# Autodesk Inventor assembly: 202.001.01_Schieberbetaetigung
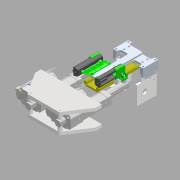
[picture p0: Inventor's stored thumbnail of the model, 180x180]
Saved by Autodesk Inventor 2021 (Build 250183000, 183)
## iProperties
Created: 2021-11-14
Part Number: 202.001.01_Schieberbetaetigung
Document SubType Name: Assembly
Designer: Oliver Ungerer
KODE_ZEICHNUNGSNUMMER: TFVEM_110M
BENENNUNG: Fuehrung Schieber
BEARBEITER_NAME: Ungerer O.
MASSE: 2.190774
PDMREV: 0.0+
PDMRL: Entwicklung
PROI_REVISION: 0
PROI_VERSION: 0+
PROI_RELEASE: Entwicklung
PTC_MODIFIED: True
PROI_CREATED_BY: Kantioler_adm
PROI_CREATED_ON: 07.03.2008 12:11:19
PROI_LOCATION: Root-Ordner/Pro_stds/Start_Files
MATERIALART: -
EINHEIT: ST
HERSTELLER_PREIS: 0.0
PRUEFER_NAME: Uo
PTC_ORGANIZATION_ID: Durst
PTC_WM_REVISION: 0
PTC_WM_ITERATION: 0
PTC_WM_VERSION: 0.0
PTC_WM_LIFECYCLE_STATE: Entwicklung
PTC_WM_LIFECYCLE: 02 Durst
PTC_WM_CREATED_BY: Oliver Ungerer (oungerer: Durst)
PTC_WM_CREATED_ON: 01.08.21
PTC_WM_MODIFIED_BY: Oliver Ungerer (oungerer: Durst)
PTC_WM_MODIFIED_ON: 01.08.21
AEND_INDEX: 0
VERSION: 0
STATUS: 0.0
Author: Oliver Ungerer
## Documents named in this file (20)
- E:\Dokumente\MCI-Mechatronik\Master\Semester_3\Projekt2_CAD\102_Vereinzelung\202.001.01_Schieberbetaetigung.iam
- E:\Dokumente\MCI-Mechatronik\Master\Semester_3\Projekt2_CAD\102_Vereinzelung\0001_IGUS_SCHIENE.ipt
- E:\Dokumente\MCI-Mechatronik\Master\Semester_3\Projekt2_CAD\102_Vereinzelung\1346134.ipt
- E:\Dokumente\MCI-Mechatronik\Master\Semester_3\Projekt2_CAD\102_Vereinzelung\TFVEM_10100.ipt
- E:\Dokumente\MCI-Mechatronik\Master\Semester_3\Projekt2_CAD\102_Vereinzelung\TFVEM_1106.ipt
- E:\Dokumente\MCI-Mechatronik\Master\Semester_3\Projekt2_CAD\102_Vereinzelung\TFVEM_1101.ipt
- E:\Dokumente\MCI-Mechatronik\Master\Semester_3\Projekt2_CAD\102_Vereinzelung\TFVEM_10102.ipt
- E:\Dokumente\MCI-Mechatronik\Master\Semester_3\Projekt2_CAD\102_Vereinzelung\TFVEM_10103.ipt
- E:\Dokumente\MCI-Mechatronik\Master\Semester_3\Projekt2_CAD\102_Vereinzelung\TFVEM_10104.ipt
- E:\Dokumente\MCI-Mechatronik\Master\Semester_3\Projekt2_CAD\102_Vereinzelung\202.001.02_Kraftlimitierung.iam
- E:\Dokumente\MCI-Mechatronik\Master\Semester_3\Projekt2_CAD\102_Vereinzelung\202.001.03_Kraftlimitierung.iam
- E:\Dokumente\MCI-Mechatronik\Master\Semester_3\Projekt2_CAD\102_Vereinzelung\CAHB-10-B1A-050158-AAAA0A-000.iam
- E:\Dokumente\MCI-Mechatronik\Master\Semester_3\Projekt2_CAD\102_Vereinzelung\TFVEM_10105.ipt
- E:\Dokumente\MCI-Mechatronik\Master\Semester_3\Projekt2_CAD\102_Vereinzelung\TFVEM_1009.ipt
- E:\Dokumente\MCI-Mechatronik\Master\Semester_3\Projekt2_CAD\102_Vereinzelung\1237347.ipt
- E:\Dokumente\MCI-Mechatronik\Master\Semester_3\Projekt2_CAD\102_Vereinzelung\1126405.ipt
- E:\Dokumente\MCI-Mechatronik\Master\Semester_3\Projekt2_CAD\102_Vereinzelung\1126767.ipt
- E:\Dokumente\MCI-Mechatronik\Master\Semester_3\Projekt2_CAD\102_Vereinzelung\202.001.04_Zapfen_Aktor.ipt
- E:\Dokumente\MCI-Mechatronik\Master\Semester_3\Projekt2_CAD\102_Vereinzelung\202.001.05_Zapfen_Aktor_Auflage.ipt
- E:\Dokumente\MCI-Mechatronik\Master\Semester_3\Projekt2_CAD\102_Vereinzelung\202.001.05_Anbindung_Aktor.ipt
## Components (31 placed, 20 different names)
1. 0001_IGUS_SCHIENE — Fluchtend:1, Passend:15, Winkel:1, Passend:20, Winkel:2, Fluchtend:2, Passend:21, Winkel:3, Passend:23, Winkel:4, Fluchtend:69, Winkel:5
2. 1346134 — Fluchtend:1, Passend:15, Winkel:1, Passend:16, Passend:17, Passend:18, Passend:19
3. 1346134:1 — Passend:22, Passend:23, Winkel:4, Passend:24, Passend:25, Passend:26
4. 1346134:2 — Fluchtend:2, Passend:21, Winkel:3, Passend:22, Passend:30, Passend:32
5. 1346134:3 — Passend:19, Passend:20, Winkel:2, Passend:31
6. TFVEM_10100 — Passend:16, Passend:17, Passend:18, Passend:27, Passend:29
7. TFVEM_1106 — Passend:27, Passend:28, Passend:29, Passend:36, Passend:37, Passend:38, Passend:48, Passend:49, Passend:50
8. TFVEM_1101 — Passend:30, Passend:31, Passend:32, Passend:33, Passend:34, Passend:35, Passend:45, Passend:46, Passend:47
9. TFVEM_10100:1 — Passend:24, Passend:25, Passend:26, Passend:28
10. TFVEM_10102 — Passend:36, Passend:37, Passend:38, Passend:42, Passend:43, Passend:44
11. TFVEM_10103 — Passend:42, Passend:43, Passend:44
12. TFVEM_10102:1 — Passend:33, Passend:34, Passend:35, Passend:39, Passend:40, Passend:41
13. TFVEM_10104 — Passend:39, Passend:40, Passend:41
14. 202.001.02_Kraftlimitierung [sub-assembly] — Passend:45, Passend:46, Passend:47, Passend:51, Passend:52, Passend:53, Passend:54
15. 202.001.03_Kraftlimitierung [sub-assembly] — Passend:48, Passend:49, Passend:50, Passend:59, Passend:60, Passend:62
16. 502.001.01_Linearaktor [sub-assembly] — Passend:1, Passend:2, Fluchtend:70, Passend:70
17. CAHB-10-B1A-050158-AAAA0A-000:2 [sub-assembly] — Fluchtend:69, Passend:67, Winkel:5, Passend:68, Passend:69, Fluchtend:70
18. TFVEM_10105 — Passend:59, Passend:60, Passend:61, Passend:63, Passend:64, Passend:65, Passend:67
19. TFVEM_1009 — Passend:51, Passend:52, Passend:55, Passend:56, Passend:57, Passend:70
20. 1237347 — Passend:55, Passend:56, Passend:58
21. 1237347:1 — Passend:63, Passend:64, Passend:66
22. 1126405 — Passend:65, Passend:66
23. 1126405:1 — Passend:57, Passend:58
24. 1126767 — Passend:53, Passend:54
25. 1126767:1 — Passend:61, Passend:62
26. 202.001.04_Zapfen_Aktor:1 — Passend:7, Passend:8, Passend:68, Passend:69
27. 202.001.04_Zapfen_Aktor:2 — Passend:1, Passend:2, Passend:5, Passend:6
28. 202.001.05_Zapfen_Aktor_Auflage:3 — Passend:7, Passend:8
29. 202.001.05_Zapfen_Aktor_Auflage:4 — Passend:5, Passend:6
30. 202.001.05_Anbindung_Aktor:1
31. 202.001.05_Anbindung_Aktor:2
## Relationships (77: Mate 68, Angle 5, Flush 4)
- Passend:1 [Mate] (1 mm): 502.001.01_Linearaktor ↔ 202.001.04_Zapfen_Aktor:2
- Passend:2 [Mate]: 502.001.01_Linearaktor ↔ 202.001.04_Zapfen_Aktor:2
- Passend:5 [Mate]: 202.001.04_Zapfen_Aktor:2 ↔ 202.001.05_Zapfen_Aktor_Auflage:4
- Passend:6 [Mate]: 202.001.04_Zapfen_Aktor:2 ↔ 202.001.05_Zapfen_Aktor_Auflage:4
- Passend:7 [Mate]: 202.001.04_Zapfen_Aktor:1 ↔ 202.001.05_Zapfen_Aktor_Auflage:3
- Passend:8 [Mate]: 202.001.04_Zapfen_Aktor:1 ↔ 202.001.05_Zapfen_Aktor_Auflage:3
- [Mate]: 202.001.04_Zapfen_Aktor:2 ↔ 202.001.05_Anbindung_Aktor:1
- [Mate]: 202.001.04_Zapfen_Aktor:2 ↔ 202.001.05_Anbindung_Aktor:1
- [Mate]: 202.001.04_Zapfen_Aktor:1 ↔ 202.001.05_Anbindung_Aktor:1
- [Mate]: 202.001.05_Zapfen_Aktor_Auflage:4 ↔ 202.001.05_Anbindung_Aktor:2
- [Mate]: 202.001.05_Zapfen_Aktor_Auflage:3 ↔ 202.001.05_Anbindung_Aktor:2
- [Mate]: 202.001.05_Zapfen_Aktor_Auflage:4 ↔ 202.001.05_Anbindung_Aktor:2
- Fluchtend:1 [Flush] (0.5 mm): 0001_IGUS_SCHIENE ↔ 1346134
- Passend:15 [Mate]: 0001_IGUS_SCHIENE ↔ 1346134
- Winkel:1 [Angle] (0 deg): 0001_IGUS_SCHIENE ↔ 1346134
- Passend:16 [Mate]: 1346134 ↔ TFVEM_10100
- Passend:17 [Mate]: 1346134 ↔ TFVEM_10100
- Passend:18 [Mate]: 1346134 ↔ TFVEM_10100
- Passend:19 [Mate] (51 mm): 1346134 ↔ 1346134:3
- Passend:20 [Mate]: 0001_IGUS_SCHIENE ↔ 1346134:3
- Winkel:2 [Angle] (0 deg): 0001_IGUS_SCHIENE ↔ 1346134:3
- Fluchtend:2 [Flush] (0.5 mm): 0001_IGUS_SCHIENE ↔ 1346134:2
- Passend:21 [Mate]: 0001_IGUS_SCHIENE ↔ 1346134:2
- Winkel:3 [Angle] (0 deg): 0001_IGUS_SCHIENE ↔ 1346134:2
- Passend:22 [Mate] (51 mm): 1346134:1 ↔ 1346134:2
- Passend:23 [Mate]: 0001_IGUS_SCHIENE ↔ 1346134:1
- Winkel:4 [Angle] (0 deg): 0001_IGUS_SCHIENE ↔ 1346134:1
- Passend:24 [Mate]: 1346134:1 ↔ TFVEM_10100:1
- Passend:25 [Mate]: 1346134:1 ↔ TFVEM_10100:1
- Passend:26 [Mate]: 1346134:1 ↔ TFVEM_10100:1
- Passend:27 [Mate]: TFVEM_10100 ↔ TFVEM_1106
- Passend:28 [Mate]: TFVEM_1106 ↔ TFVEM_10100:1
- Passend:29 [Mate]: TFVEM_10100 ↔ TFVEM_1106
- Passend:30 [Mate]: 1346134:2 ↔ TFVEM_1101
- Passend:31 [Mate]: 1346134:3 ↔ TFVEM_1101
- Passend:32 [Mate]: 1346134:2 ↔ TFVEM_1101
- Passend:33 [Mate]: TFVEM_1101 ↔ TFVEM_10102:1
- Passend:34 [Mate]: TFVEM_1101 ↔ TFVEM_10102:1
- Passend:35 [Mate]: TFVEM_1101 ↔ TFVEM_10102:1
- Passend:36 [Mate]: TFVEM_1106 ↔ TFVEM_10102
- Passend:37 [Mate]: TFVEM_1106 ↔ TFVEM_10102
- Passend:38 [Mate]: TFVEM_1106 ↔ TFVEM_10102
- Passend:39 [Mate]: TFVEM_10102:1 ↔ TFVEM_10104
- Passend:40 [Mate]: TFVEM_10102:1 ↔ TFVEM_10104
- Passend:41 [Mate]: TFVEM_10102:1 ↔ TFVEM_10104
- Passend:42 [Mate]: TFVEM_10102 ↔ TFVEM_10103
- Passend:43 [Mate]: TFVEM_10102 ↔ TFVEM_10103
- Passend:44 [Mate]: TFVEM_10102 ↔ TFVEM_10103
- Passend:45 [Mate]: TFVEM_1101 ↔ 202.001.02_Kraftlimitierung
- Passend:46 [Mate]: TFVEM_1101 ↔ 202.001.02_Kraftlimitierung
- Passend:47 [Mate]: TFVEM_1101 ↔ 202.001.02_Kraftlimitierung
- Passend:48 [Mate]: TFVEM_1106 ↔ 202.001.03_Kraftlimitierung
- Passend:49 [Mate]: TFVEM_1106 ↔ 202.001.03_Kraftlimitierung
- Passend:50 [Mate]: TFVEM_1106 ↔ 202.001.03_Kraftlimitierung
- Passend:51 [Mate]: 202.001.02_Kraftlimitierung ↔ TFVEM_1009
- Passend:52 [Mate]: 202.001.02_Kraftlimitierung ↔ TFVEM_1009
- Passend:53 [Mate]: 202.001.02_Kraftlimitierung ↔ 1126767
- Passend:54 [Mate]: 202.001.02_Kraftlimitierung ↔ 1126767
- Passend:55 [Mate]: TFVEM_1009 ↔ 1237347
- Passend:56 [Mate]: TFVEM_1009 ↔ 1237347
- Passend:57 [Mate]: TFVEM_1009 ↔ 1126405:1
- Passend:58 [Mate]: 1237347 ↔ 1126405:1
- Passend:59 [Mate]: 202.001.03_Kraftlimitierung ↔ TFVEM_10105
- Passend:60 [Mate]: 202.001.03_Kraftlimitierung ↔ TFVEM_10105
- Passend:61 [Mate]: TFVEM_10105 ↔ 1126767:1
- Passend:62 [Mate]: 202.001.03_Kraftlimitierung ↔ 1126767:1
- Passend:63 [Mate]: TFVEM_10105 ↔ 1237347:1
- Passend:64 [Mate]: TFVEM_10105 ↔ 1237347:1
- Passend:65 [Mate]: TFVEM_10105 ↔ 1126405
- Passend:66 [Mate]: 1237347:1 ↔ 1126405
- Fluchtend:69 [Flush] (6 mm): 0001_IGUS_SCHIENE ↔ CAHB-10-B1A-050158-AAAA0A-000:2
- Passend:67 [Mate]: CAHB-10-B1A-050158-AAAA0A-000:2 ↔ TFVEM_10105
- Winkel:5 [Angle] (0 deg): 0001_IGUS_SCHIENE ↔ CAHB-10-B1A-050158-AAAA0A-000:2
- Passend:68 [Mate]: CAHB-10-B1A-050158-AAAA0A-000:2 ↔ 202.001.04_Zapfen_Aktor:1
- Passend:69 [Mate] (1 mm): CAHB-10-B1A-050158-AAAA0A-000:2 ↔ 202.001.04_Zapfen_Aktor:1
- Fluchtend:70 [Flush]: 502.001.01_Linearaktor ↔ CAHB-10-B1A-050158-AAAA0A-000:2
- Passend:70 [Mate]: 502.001.01_Linearaktor ↔ TFVEM_1009
## Named parameters: d8_d2 = 0 mm, d9_d3 = 0 mm, d10_d4 = 0 mm, d11_d6 = 0 mm, d12_d7 = 0 mm
